# Autodesk Inventor assembly: test_asm
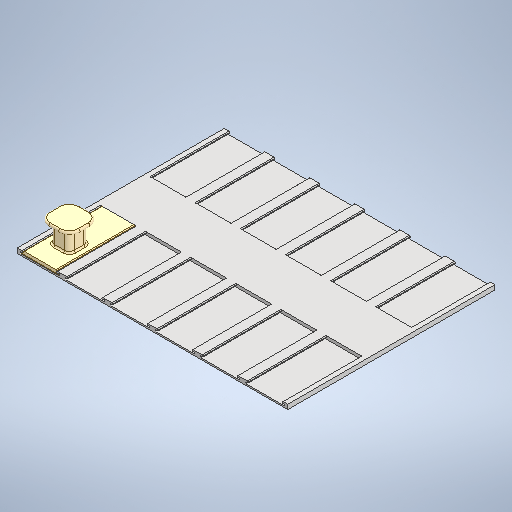
[picture p0: Inventor's stored thumbnail of the model, 512x512]
Saved by Autodesk Inventor 2025 (Build 290162000, 162)
## iProperties
Created: 2025-01-15
Part Number: test_asm
Document SubType Name: Assembly
Designer: ethan
Author: ethan
## Documents named in this file (3)
- C:\Users\ethan\OneDrive\Documents\GitHub\3D-Pants\CordManage\test_asm.iam
- C:\Users\ethan\OneDrive\Documents\GitHub\3D-Pants\CordManage\Holder.ipt
- C:\Users\ethan\OneDrive\Documents\GitHub\3D-Pants\CordManage\Insert.ipt
## Components (2 placed, 2 different names)
1. Holder:1 — Mate:1, Mate:2
2. Insert:1 — Mate:1, Mate:2
## Relationships (2: Mate 2)
- Mate:1: Holder:1 ↔ Insert:1
- Mate:2: Holder:1 ↔ Insert:1
